# Autodesk Inventor assembly: BodyAssembly
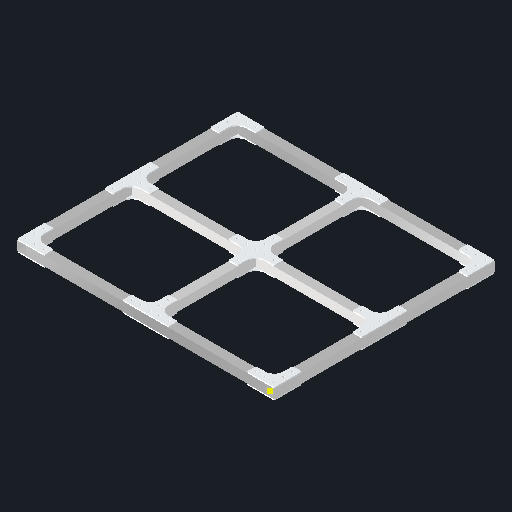
[picture p0: Inventor's stored thumbnail of the model, 512x512]
Saved by Autodesk Inventor 2026.1 (Build 301233020, 233B)
## iProperties
Created: 2023-09-27
Part Number: BodyAssembly
Document SubType Name: Assembly
Designer: Megan
Author: Megan
## Documents named in this file (8)
- C:\Users\t205b\OneDrive\Documents\Github\BehrendURCMechanical\CAD\Chassis V3\Body\BodyAssembly.iam
- C:\Users\t205b\OneDrive\Documents\Github\BehrendURCMechanical\CAD\Chassis V3\Body\24inTube.ipt
- C:\Users\t205b\OneDrive\Documents\Github\BehrendURCMechanical\CAD\Chassis V3\Body\26inTube.ipt
- C:\Users\t205b\OneDrive\Documents\Github\BehrendURCMechanical\CAD\Chassis V3\Body\12.5inTube.ipt
- C:\Users\t205b\OneDrive\Documents\Github\BehrendURCMechanical\CAD\Chassis V3\Body\am-3860 90 Gusset REV2.ipt
- C:\Users\t205b\OneDrive\Documents\Github\BehrendURCMechanical\CAD\Chassis V3\Body\am-4159 1IN Quad Gusset.ipt
- C:\Users\t205b\OneDrive\Documents\Github\BehrendURCMechanical\CAD\Chassis V3\Body\am-4158 1IN Tee Gusset.ipt
- C:\Users\t205b\OneDrive\Documents\Github\BehrendURCMechanical\CAD\Chassis V3\Body\22inTube.ipt
## Components (25 placed, 8 different names)
1. 24inTube:1 — Mate:1, Flush:1, Flush:2, Mate:2, Flush:3, Flush:4, Flush:16, Mate:12, Flush:18, Mate:13, Flush:21, Flush:22, Mate:14, Mate:23, Mate:24, Flush:43, Flush:49, Flush:61
2. 24inTube:2 — Mate:3, Flush:5, Flush:6, Flush:10, Mate:9, Flush:12, Mate:10, Flush:15, Mate:15, Flush:25, Mate:16, Flush:27, Mate:19, Flush:32, Mate:20, Flush:34, Mate:32
3. 26inTube:1 — Mate:1, Flush:1, Flush:2, Mate:3, Flush:5, Flush:6, Flush:20, Flush:23, Flush:24, Flush:26, Mate:25, Flush:44, Flush:47, Mate:30
4. 26inTube:2 — Mate:2, Flush:3, Flush:4, Flush:13, Flush:14, Mate:11, Flush:17, Flush:19, Mate:21, Flush:37, Mate:22, Flush:38, Mate:27, Mate:35
5. 13inTube:2 — Flush:10, Flush:33, Flush:35, Mate:28, Mate:32, Mate:33, Flush:51, Flush:54, Mate:35
6. am-3860 90 Gusset REV2:1 — Mate:9, Flush:12, Flush:13
7. am-3860 90 Gusset REV2:2 — Mate:10, Flush:14, Flush:15
8. am-3860 90 Gusset REV2:3 — Mate:11, Flush:16, Flush:17
9. am-3860 90 Gusset REV2:4 — Mate:12, Flush:18, Flush:19
10. am-3860 90 Gusset REV2:5 — Mate:15, Flush:24, Flush:25
11. am-3860 90 Gusset REV2:6 — Mate:16, Flush:26, Flush:27
12. am-3860 90 Gusset REV2:7 — Mate:13, Flush:20, Flush:21
13. am-3860 90 Gusset REV2:8 — Flush:22, Flush:23, Mate:14
14. am-4159 1IN Quad Gusset:1 — Mate:33, Flush:52, Flush:53
15. am-4159 1IN Quad Gusset:2 — Flush:54, Flush:55, Mate:34
16. am-4158 1IN Tee Gusset:1 — Mate:19, Flush:32, Flush:33
17. am-4158 1IN Tee Gusset:2 — Mate:20, Flush:34, Flush:35
18. am-4158 1IN Tee Gusset:3 — Mate:21, Flush:37, Flush:59
19. am-4158 1IN Tee Gusset:4 — Mate:22, Flush:38, Flush:58
20. am-4158 1IN Tee Gusset:5 — Mate:23, Flush:60, Flush:61
21. am-4158 1IN Tee Gusset:6 — Mate:24, Flush:43, Flush:50
22. am-4158 1IN Tee Gusset:7 — Mate:25, Flush:44, Mate:26, Flush:57
23. am-4158 1IN Tee Gusset:8 — Flush:47, Mate:30, Flush:56
24. 12.5inTube:5 — Flush:49, Mate:31, Flush:50, Flush:51, Flush:52, Flush:60
25. 22inTube:1 — Mate:26, Mate:27, Mate:28, Mate:31, Flush:53, Flush:55, Mate:34, Flush:56, Flush:57, Flush:58, Flush:59
## Relationships (72: Flush 45, Mate 27)
- Mate:1: 24inTube:1 ↔ 26inTube:1
- Flush:1: 24inTube:1 ↔ 26inTube:1
- Flush:2: 24inTube:1 ↔ 26inTube:1
- Mate:2: 24inTube:1 ↔ 26inTube:2
- Flush:3: 24inTube:1 ↔ 26inTube:2
- Flush:4: 24inTube:1 ↔ 26inTube:2
- Mate:3: 24inTube:2 ↔ 26inTube:1
- Flush:5: 24inTube:2 ↔ 26inTube:1
- Flush:6: 24inTube:2 ↔ 26inTube:1
- Flush:10: 24inTube:2 ↔ 13inTube:2
- Mate:9: 24inTube:2 ↔ am-3860 90 Gusset REV2:1
- Flush:12: 24inTube:2 ↔ am-3860 90 Gusset REV2:1
- Flush:13: 26inTube:2 ↔ am-3860 90 Gusset REV2:1
- Mate:10: 24inTube:2 ↔ am-3860 90 Gusset REV2:2
- Flush:14: 26inTube:2 ↔ am-3860 90 Gusset REV2:2
- Flush:15: 24inTube:2 ↔ am-3860 90 Gusset REV2:2
- Mate:11: 26inTube:2 ↔ am-3860 90 Gusset REV2:3
- Flush:16: 24inTube:1 ↔ am-3860 90 Gusset REV2:3
- Flush:17: 26inTube:2 ↔ am-3860 90 Gusset REV2:3
- Mate:12: 24inTube:1 ↔ am-3860 90 Gusset REV2:4
- Flush:18: 24inTube:1 ↔ am-3860 90 Gusset REV2:4
- Flush:19: 26inTube:2 ↔ am-3860 90 Gusset REV2:4
- Mate:13: 24inTube:1 ↔ am-3860 90 Gusset REV2:7
- Flush:20: 26inTube:1 ↔ am-3860 90 Gusset REV2:7
- Flush:21: 24inTube:1 ↔ am-3860 90 Gusset REV2:7
- Flush:22: 24inTube:1 ↔ am-3860 90 Gusset REV2:8
- Flush:23: 26inTube:1 ↔ am-3860 90 Gusset REV2:8
- Mate:14: 24inTube:1 ↔ am-3860 90 Gusset REV2:8
- Mate:15: 24inTube:2 ↔ am-3860 90 Gusset REV2:5
- Flush:24: 26inTube:1 ↔ am-3860 90 Gusset REV2:5
- Flush:25: 24inTube:2 ↔ am-3860 90 Gusset REV2:5
- Mate:16: 24inTube:2 ↔ am-3860 90 Gusset REV2:6
- Flush:26: 26inTube:1 ↔ am-3860 90 Gusset REV2:6
- Flush:27: 24inTube:2 ↔ am-3860 90 Gusset REV2:6
- Mate:19: 24inTube:2 ↔ am-4158 1IN Tee Gusset:1
- Flush:32: 24inTube:2 ↔ am-4158 1IN Tee Gusset:1
- Flush:33: 13inTube:2 ↔ am-4158 1IN Tee Gusset:1
- Mate:20: 24inTube:2 ↔ am-4158 1IN Tee Gusset:2
- Flush:34: 24inTube:2 ↔ am-4158 1IN Tee Gusset:2
- Flush:35: 13inTube:2 ↔ am-4158 1IN Tee Gusset:2
- Mate:21: 26inTube:2 ↔ am-4158 1IN Tee Gusset:3
- Flush:37: 26inTube:2 ↔ am-4158 1IN Tee Gusset:3
- Mate:22: 26inTube:2 ↔ am-4158 1IN Tee Gusset:4
- Flush:38: 26inTube:2 ↔ am-4158 1IN Tee Gusset:4
- Mate:23: 24inTube:1 ↔ am-4158 1IN Tee Gusset:5
- Mate:24: 24inTube:1 ↔ am-4158 1IN Tee Gusset:6
- Flush:43: 24inTube:1 ↔ am-4158 1IN Tee Gusset:6
- Mate:25: 26inTube:1 ↔ am-4158 1IN Tee Gusset:7
- Flush:44: 26inTube:1 ↔ am-4158 1IN Tee Gusset:7
- Flush:47: 26inTube:1 ↔ am-4158 1IN Tee Gusset:8
- Mate:26: am-4158 1IN Tee Gusset:7 ↔ 22inTube:1
- Mate:27: 26inTube:2 ↔ 22inTube:1
- Mate:28: 13inTube:2 ↔ 22inTube:1
- Flush:49: 24inTube:1 ↔ 12.5inTube:5
- Mate:30: 26inTube:1 ↔ am-4158 1IN Tee Gusset:8
- Mate:31: 12.5inTube:5 ↔ 22inTube:1
- Mate:32: 24inTube:2 ↔ 13inTube:2
- Mate:33: 13inTube:2 ↔ am-4159 1IN Quad Gusset:1
- Flush:50: am-4158 1IN Tee Gusset:6 ↔ 12.5inTube:5
- Flush:51: 13inTube:2 ↔ 12.5inTube:5
- Flush:52: am-4159 1IN Quad Gusset:1 ↔ 12.5inTube:5
- Flush:53: am-4159 1IN Quad Gusset:1 ↔ 22inTube:1
- Flush:54: 13inTube:2 ↔ am-4159 1IN Quad Gusset:2
- Flush:55: am-4159 1IN Quad Gusset:2 ↔ 22inTube:1
- Mate:34: am-4159 1IN Quad Gusset:2 ↔ 22inTube:1
- Flush:56: am-4158 1IN Tee Gusset:8 ↔ 22inTube:1
- Flush:57: am-4158 1IN Tee Gusset:7 ↔ 22inTube:1
- Flush:58: am-4158 1IN Tee Gusset:4 ↔ 22inTube:1
- Flush:59: am-4158 1IN Tee Gusset:3 ↔ 22inTube:1
- Flush:60: am-4158 1IN Tee Gusset:5 ↔ 12.5inTube:5
- Flush:61: 24inTube:1 ↔ am-4158 1IN Tee Gusset:5
- Mate:35 (266.7 mm): 26inTube:2 ↔ 13inTube:2
